# Autodesk Inventor assembly: Dual 775pro_0_1-2inHex
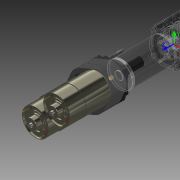
[picture p0: Inventor's stored thumbnail of the model, 180x180]
Saved by Autodesk Inventor 2022 (Build 260153000, 153)
## iProperties
Created: 2018-08-19
Part Number: Dual 775pro_0_1-2inHex
Document SubType Name: Assembly
Mass: 1123.04 g
Surface Area: 1203.25 cm^2
Volume: 285.054 cm^3
Density: 3.93975 g/cm^3
## Documents named in this file (9)
- C:\Users\Cal\Desktop\Robotics\Design\Collaborative\Collaborative Parts Library\General Gearboxes\Planetaries\Versaplanetary\VersaPlanetary\Dual 775pro, 0 Stages, 1-2in Hex Output.iam
- C:\Users\Cal\Desktop\Robotics\Design\Collaborative\Collaborative Parts Library\General Gearboxes\Planetaries\Versaplanetary\Screws\8-32 x 0.75in Screw.ipt
- C:\Users\Cal\Desktop\Robotics\Design\Collaborative\Collaborative Parts Library\Power Transfer\Bearings and Bushings\Bearings\6902ZZ.ipt
- E:\Middleton Robotics\Collaborative Robots\Colaborative Part Library\General Gearboxes\Planetaries\Versaplanetary\V2 Stages\V2 Output Stage.iam
- E:\Middleton Robotics\Collaborative Robots\Colaborative Part Library\General Gearboxes\Planetaries\Versaplanetary\V2 Stages\Dual Input Stage.iam
- E:\Middleton Robotics\Collaborative Robots\Collaborative Part Library\Power Transfer\Bearings.ipt
- C:\Users\Cal\Desktop\Robotics\Design\Collaborative\Collaborative Parts Library\General Gearboxes\Planetaries\Versaplanetary\V2 Stages\V2 Output Stage\VP V2 Output Stage 1-2in Hex.iam
- C:\Users\Cal\Desktop\Robotics\Design\Collaborative\Collaborative Parts Library\General Gearboxes\Planetaries\Versaplanetary\V2 Stages\Dual Input Stage\VP Dual 775pro Input.iam
- C:\Users\Cal\Desktop\Robotics\Design\Collaborative\Collaborative Parts Library\General Gearboxes\Planetaries\Versaplanetary\VersaPlanetary.iam
## Components (6 placed, 4 different names)
1. VP V2 Output Stage 1-2in Hex:1 [sub-assembly] — 0StageDualInputMate1, 0StageDualInputMate2, 0StageDualInputMate3, Insert:25
2. VP Dual 775pro Input:1 [sub-assembly] — 0StageDualInputMate1, 0StageDualInputMate2, 0StageDualInputMate3, Insert:16, Insert:17
3. 8-32 x 0.75in Screw:1 — Insert:16
4. 8-32 x 0.75in Screw:2 — Insert:17
5. 6902ZZ:1
6. 6902ZZ:2 — Insert:25
## Relationships (6: Mate 3, Insert 3)
- 0StageDualInputMate1 [Mate]: VP V2 Output Stage 1-2in Hex:1 ↔ VP Dual 775pro Input:1
- 0StageDualInputMate2 [Mate]: VP V2 Output Stage 1-2in Hex:1 ↔ VP Dual 775pro Input:1
- 0StageDualInputMate3 [Mate]: VP V2 Output Stage 1-2in Hex:1 ↔ VP Dual 775pro Input:1
- Insert:16: VP Dual 775pro Input:1 ↔ 8-32 x 0.75in Screw:1
- Insert:17: VP Dual 775pro Input:1 ↔ 8-32 x 0.75in Screw:2
- Insert:25: VP V2 Output Stage 1-2in Hex:1 ↔ 6902ZZ:2
